# Autodesk Inventor assembly: Ensamble Prueba
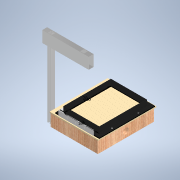
[picture p0: Inventor's stored thumbnail of the model, 180x180]
Saved by Autodesk Inventor 2022.6 (Build 266554000, 554)
## iProperties
Created: 2025-01-16
Part Number: Ensamble Prueba
Document SubType Name: Assembly
Designer: johan
Author: johan
## Documents named in this file (9)
- D:\RutasNew\Desktop\Desktop\Ensamble Prueba.iam
- D:\RutasNew\Desktop\Desktop\MADERA.ipt
- D:\RutasNew\Desktop\Desktop\Fomi.ipt
- D:\RutasNew\Desktop\Desktop\rejilla.ipt
- D:\RutasNew\Desktop\Desktop\Tapa Superior.ipt
- D:\RutasNew\Desktop\Desktop\Tapa Inferior.ipt
- D:\RutasNew\Desktop\Desktop\Pestaña.ipt
- D:\RutasNew\Desktop\Desktop\Perfil400mm.ipt
- D:\RutasNew\Desktop\Desktop\Travesaño.ipt
## Components (8 placed, 8 different names)
1. MADERA:1 — Coincidencia:1, Nivelación:1, Nivelación:2
2. Fomi:1 — Coincidencia:1, Nivelación:1, Nivelación:2, Coincidencia:2
3. rejilla:1 — Coincidencia:2, Coincidencia:4, Nivelación:5
4. Tapa Superior:1 — Coincidencia:3, Nivelación:3, Nivelación:4
5. Tapa Inferior:1 — Coincidencia:3, Nivelación:3, Nivelación:4, Coincidencia:4, Nivelación:5
6. Pestaña:2
7. Perfil400mm:4 — Nivelación:6
8. Travesaño:1 — Nivelación:6
## Relationships (10: Flush 6, Mate 4)
- Coincidencia:1 [Mate]: MADERA:1 ↔ Fomi:1
- Nivelación:1 [Flush]: MADERA:1 ↔ Fomi:1
- Nivelación:2 [Flush]: MADERA:1 ↔ Fomi:1
- Coincidencia:2 [Mate]: Fomi:1 ↔ rejilla:1
- Coincidencia:3 [Mate]: Tapa Superior:1 ↔ Tapa Inferior:1
- Nivelación:3 [Flush]: Tapa Superior:1 ↔ Tapa Inferior:1
- Nivelación:4 [Flush]: Tapa Superior:1 ↔ Tapa Inferior:1
- Coincidencia:4 [Mate]: rejilla:1 ↔ Tapa Inferior:1
- Nivelación:5 [Flush]: rejilla:1 ↔ Tapa Inferior:1
- Nivelación:6 [Flush]: Perfil400mm:4 ↔ Travesaño:1
